# Autodesk Inventor assembly: 20-705
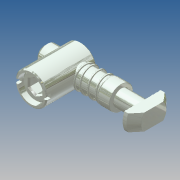
[picture p0: Inventor's stored thumbnail of the model, 180x180]
Saved by Autodesk Inventor 2011 SP2 (Build 150309200, 309)
## iProperties
Created: 2011-01-07
Part Number: 20-705
Document SubType Name: Assembly
Designer: dc85560
Stock Number: 20-705
Mass: 6.47254 g
Surface Area: 49.745 cm^2
Volume: 6.47254 cm^3
Density: 1 g/cm^3
Translation Standard: STEP AP214IS
File Name: 099b081511s.STEP
Preprocessor: SolidWorks 2010
Postprocessor: Build: 320, Release: 2008 SP2 - Date: Mon 11/26/2007
Sent Units: MILLIMETERS
Uncertainty: 1e-05
Title: Central Connector Parallel
Author: dc85560
## Documents named in this file (5)
- R:\PSD 3 Library Update\IPS Part Files\02-Fasteners\06-Central Connector\20-705.iam
- R:\PSD 3 Library Update\IPS Part Files\02-Fasteners\06-Central Connector\20-705Z3.ipt
- R:\PSD 3 Library Update\IPS Part Files\02-Fasteners\06-Central Connector\20-705Z1.ipt
- R:\PSD 3 Library Update\IPS Part Files\02-Fasteners\06-Central Connector\20-705Z2.ipt
- R:\PSD 3 Library Update\IPS Part Files\02-Fasteners\06-Central Connector\20-705Z4.ipt
## Components (4 placed, 4 different names)
1. 20-705Z3:1
2. 20-705Z1:1 — Mate:1, Flush:1
3. 20-705Z2:1 — Angle:1
4. 20-705Z4:1 — Mate:1, Angle:1, Flush:1
## Relationships (3: Mate 1, Angle 1, Flush 1)
- Mate:1: 20-705Z1:1 ↔ 20-705Z4:1
- Angle:1 (0 deg): 20-705Z2:1 ↔ 20-705Z4:1
- Flush:1: 20-705Z1:1 ↔ 20-705Z4:1
